# Autodesk Inventor assembly: AL_plate_600x460x2t_door
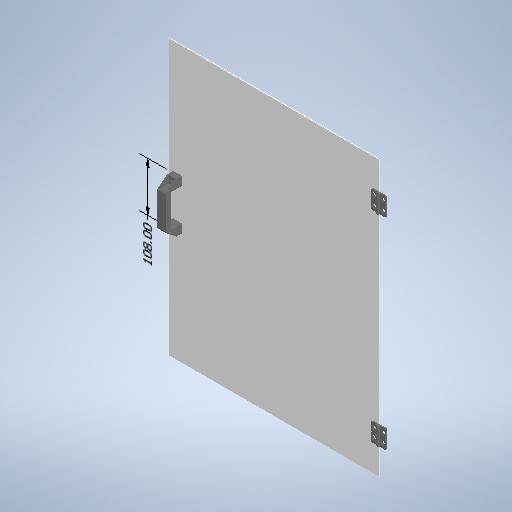
[picture p0: Inventor's stored thumbnail of the model, 512x512]
Saved by Autodesk Inventor 2025.4 (Build 294407000, 407)
## iProperties
Created: 2026-06-10
Part Number: AL_plate_600x460x2t_door
Document SubType Name: Assembly
Designer: dalbi
Author: dalbi
## Documents named in this file (4)
- C:\Users\dalbi\OneDrive\바탕 화면\트리보 설계파일\stl\AL_plate_600x460x2t_door.iam
- C:\Users\dalbi\OneDrive\바탕 화면\트리보 설계파일\최종 설계 파일(조립시 참고할 파일)\AL_Plate_Outer_600X460X2t.ipt
- C:\Users\dalbi\OneDrive\바탕 화면\트리보 설계파일\최종 설계 파일(조립시 참고할 파일)\Handle.ipt
- C:\Users\dalbi\OneDrive\바탕 화면\트리보 설계파일\최종 설계 파일(조립시 참고할 파일)\Plastic_Hinge.ipt
## Components (6 placed, 3 different names)
1. AL_Plate_Outer_600X460X2t:1 — 메이트:1, 메이트:2, 플러쉬:1, 플러쉬:2, 메이트:3, 플러쉬:3, 메이트:4, 메이트:7, 플러쉬:6, 메이트:8
2. Handle:1 — 메이트:1, 플러쉬:1, 플러쉬:2
3. Plastic_Hinge:1 — 메이트:2, 메이트:3, 플러쉬:3, 메이트:5, 플러쉬:4
4. Plastic_Hinge:2 — 메이트:4, 메이트:5, 플러쉬:4
5. Plastic_Hinge:3 — 메이트:7, 플러쉬:6, 메이트:8
6. Plastic_Hinge:4
## Relationships (14: Mate 8, Flush 6)
- 메이트:1 [Mate]: AL_Plate_Outer_600X460X2t:1 ↔ Handle:1
- 메이트:2 [Mate]: AL_Plate_Outer_600X460X2t:1 ↔ Plastic_Hinge:1
- 플러쉬:1 [Flush] (246 mm): AL_Plate_Outer_600X460X2t:1 ↔ Handle:1
- 플러쉬:2 [Flush] (10 mm): AL_Plate_Outer_600X460X2t:1 ↔ Handle:1
- 메이트:3 [Mate] (-15 mm): AL_Plate_Outer_600X460X2t:1 ↔ Plastic_Hinge:1
- 플러쉬:3 [Flush] (80 mm): AL_Plate_Outer_600X460X2t:1 ↔ Plastic_Hinge:1
- 메이트:4 [Mate]: AL_Plate_Outer_600X460X2t:1 ↔ Plastic_Hinge:2
- 메이트:5 [Mate]: Plastic_Hinge:1 ↔ Plastic_Hinge:2
- 플러쉬:4 [Flush]: Plastic_Hinge:1 ↔ Plastic_Hinge:2
- [Mate]: Plastic_Hinge:3 ↔ Plastic_Hinge:4
- [Flush]: Plastic_Hinge:3 ↔ Plastic_Hinge:4
- 메이트:7 [Mate]: AL_Plate_Outer_600X460X2t:1 ↔ Plastic_Hinge:3
- 플러쉬:6 [Flush] (60 mm): AL_Plate_Outer_600X460X2t:1 ↔ Plastic_Hinge:3
- 메이트:8 [Mate] (-15 mm): AL_Plate_Outer_600X460X2t:1 ↔ Plastic_Hinge:3
## Named parameters: d13_d11 = 0 mm, d14_d12 = 0 mm
